# Autodesk Inventor assembly: NewFinalAssembly
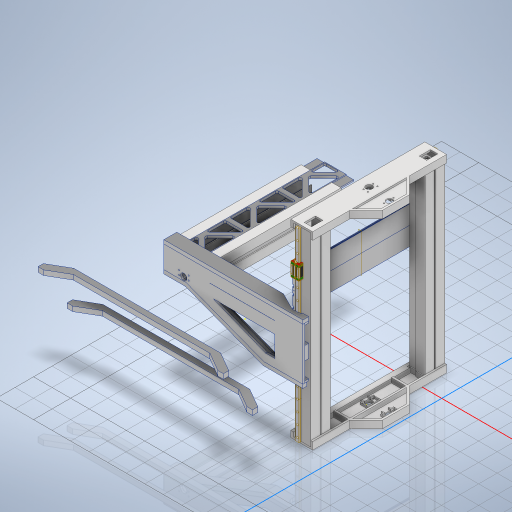
[picture p0: Inventor's stored thumbnail of the model, 512x512]
Saved by Autodesk Inventor 2024 (Build 280153000, 153)
## iProperties
Created: 2023-06-18
Part Number: NewFinalAssembly
Document SubType Name: Assembly
Designer: KirikDK
Author: KirikDK
## Documents named in this file (5)
- C:\Users\KirikDK\Documents\Stanok2023\NewFinalAssembly.iam
- C:\Users\KirikDK\Documents\Stanok2023\Xaxis.iam
- C:\Users\KirikDK\Documents\Stanok2023\HGH20_block.ipt
- C:\Users\KirikDK\Documents\Stanok2023\YaxisNew.iam
- C:\Users\KirikDK\Documents\Stanok2023\UcreplenieX.ipt
## Components (8 placed, 4 different names)
1. Xaxis:1 [sub-assembly] — Flush:1, Flush:2, Flush:3, Flush:4, Flush:5, Flush:6, Flush:7, Flush:8
2. HGH20_block:1 — Flush:1, Flush:2, Flush:9
3. HGH20_block:2 — Flush:3, Flush:4
4. HGH20_block:3 — Flush:7, Flush:8
5. HGH20_block:4 — Flush:5, Flush:6
6. YaxisNew:1 [sub-assembly] — Flush:9
7. UcreplenieX:1
8. UcreplenieX:2
## Relationships (9: Flush 9)
- Flush:1: Xaxis:1 ↔ HGH20_block:1
- Flush:2: Xaxis:1 ↔ HGH20_block:1
- Flush:3: Xaxis:1 ↔ HGH20_block:2
- Flush:4: Xaxis:1 ↔ HGH20_block:2
- Flush:5: Xaxis:1 ↔ HGH20_block:4
- Flush:6: Xaxis:1 ↔ HGH20_block:4
- Flush:7: Xaxis:1 ↔ HGH20_block:3
- Flush:8: Xaxis:1 ↔ HGH20_block:3
- Flush:9: HGH20_block:1 ↔ YaxisNew:1
